# Autodesk Inventor assembly: RearPanel
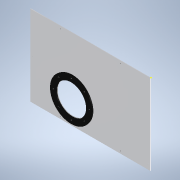
[picture p0: Inventor's stored thumbnail of the model, 180x180]
Saved by Autodesk Inventor 2020 (Build 240168000, 168)
## iProperties
Created: 2019-11-06
Part Number: RearPanel
Document SubType Name: Assembly
Designer: nicoc
Author: nicoc
## Documents named in this file (3)
- D:\Repos\P5-AIonFPGA\cad\RearPanel\RearPanel.iam
- D:\Repos\P5-AIonFPGA\cad\RearPanel\RearPanel.ipt
- D:\Repos\P5-AIonFPGA\cad\RearPanel\MountingRing.ipt
## Components (2 placed, 2 different names)
1. RearPanel:1 — Mate:1, Insert:1
2. MountingRing:1 — Mate:1, Insert:1
## Relationships (2: Mate 1, Insert 1)
- Mate:1: RearPanel:1 ↔ MountingRing:1
- Insert:1: RearPanel:1 ↔ MountingRing:1
